# Autodesk Inventor assembly: Watch Assembly
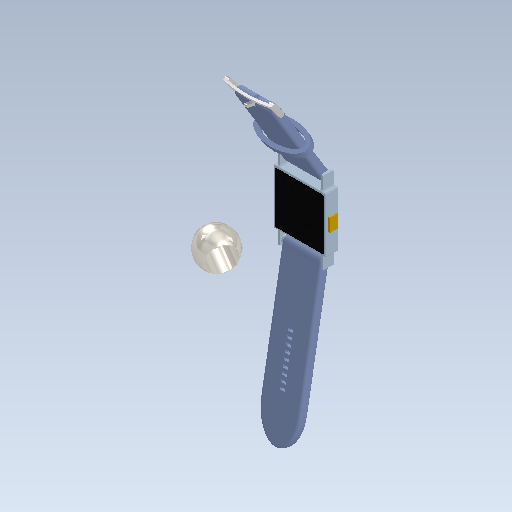
[picture p0: Inventor's stored thumbnail of the model, 512x512]
Saved by Autodesk Inventor 2020 (Build 240168000, 168)
## iProperties
Created: 2020-05-08
Part Number: Watch Assembly
Document SubType Name: Assembly
Designer: harry
Author: harry
## Documents named in this file (8)
- C:\Users\harry\OneDrive\Documents\College\Engineering\Engineering Final\Watch Assembly.iam
- C:\Users\harry\OneDrive\Documents\College\Engineering\Engineering Final\3D sketches\Smart watch Screen.ipt
- C:\Users\harry\OneDrive\Documents\College\Engineering\Engineering Final\3D sketches\Top Watch Strap.ipt
- C:\Users\harry\OneDrive\Documents\College\Engineering\Engineering Final\3D sketches\Watch bottom strap.ipt
- C:\Users\harry\OneDrive\Documents\College\Engineering\Engineering Final\3D sketches\Watch Top strap attachment.ipt
- C:\Users\harry\OneDrive\Documents\College\Engineering\Engineering Final\3D sketches\Strap band.ipt
- C:\Users\harry\OneDrive\Documents\College\Engineering\Engineering Final\3D sketches\Smart Ring.ipt
- C:\Users\harry\OneDrive\Documents\College\Engineering\Engineering Final\3D sketches\Strap holder.ipt
## Components (7 placed, 7 different names)
1. Smart watch Screen:1 — Mate:1, Mate:2, Flush:1, Mate:3
2. Top Watch Strap:1 — Mate:1, Mate:3, Mate:6, Mate:7, Mate:11, Mate:13
3. Watch bottom strap:1 — Mate:2, Flush:1
4. Watch Top strap attachment:1 — Mate:6, Mate:7, Flush:2, Mate:14, Flush:3
5. Strap band:1 — Mate:11, Mate:13, Flush:2
6. Smart Ring:1
7. Strap holder:1 — Mate:14, Flush:3
## Relationships (11: Mate 8, Flush 3)
- Mate:1: Smart watch Screen:1 ↔ Top Watch Strap:1
- Mate:2: Smart watch Screen:1 ↔ Watch bottom strap:1
- Flush:1: Smart watch Screen:1 ↔ Watch bottom strap:1
- Mate:3: Smart watch Screen:1 ↔ Top Watch Strap:1
- Mate:6: Top Watch Strap:1 ↔ Watch Top strap attachment:1
- Mate:7: Top Watch Strap:1 ↔ Watch Top strap attachment:1
- Mate:11: Top Watch Strap:1 ↔ Strap band:1
- Mate:13: Top Watch Strap:1 ↔ Strap band:1
- Flush:2: Watch Top strap attachment:1 ↔ Strap band:1
- Mate:14: Watch Top strap attachment:1 ↔ Strap holder:1
- Flush:3: Watch Top strap attachment:1 ↔ Strap holder:1
